# Autodesk Inventor assembly: Сборка
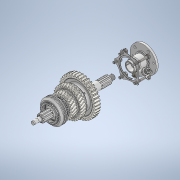
[picture p0: Inventor's stored thumbnail of the model, 180x180]
Saved by Autodesk Inventor 2021 (Build 250183000, 183)
## iProperties
Created: 2021-04-26
Part Number: Сборка
Document SubType Name: Assembly
Designer: Данил
Author: Данил
## Documents named in this file (29)
- C:\Users\Данил\Desktop\Коробка передач\Детали\Сборка.iam
- C:\Users\Данил\Desktop\Коробка передач\Детали\66-67. Картер коробки передач.ipt
- C:\Users\Данил\Desktop\Коробка передач\Детали\74. Вал первичный в сборе.iam
- C:\Users\Данил\Desktop\Коробка передач\Детали\Подшипник 180209 ГОСТ 8882-75.ipt
- C:\Users\Данил\Desktop\Коробка передач\Детали\65. Кольцо упорное подшипника.ipt
- C:\Users\Данил\Desktop\Коробка передач\Детали\76. Гайка первичного вала.ipt
- C:\Users\Данил\Desktop\Коробка передач\Детали\75. Прокладка крышки.ipt
- C:\Users\Данил\Desktop\Коробка передач\Детали\73. Крышка подшипника.ipt
- C:\Users\Данил\Desktop\Коробка передач\Детали\34. Скоба оттяжной пружины муфты.ipt
- C:\Users\Данил\Documents\Inventor\Content Center Files\R2021\ru-RU\GOST 6402-70\Шайба  8 L ГОСТ 6402-70.ipt
- C:\Users\Данил\Documents\Inventor\Content Center Files\R2021\ru-RU\Bolt GOST 7798-78\Болт M8-6g×22(S13) ГОСТ 7798-70.ipt
- C:\Users\Данил\Desktop\Коробка передач\Детали\73. Вал вторичный в сборе.iam
- C:\Users\Данил\Desktop\Коробка передач\Детали\64. Кольцо блокирующее.ipt
- C:\Users\Данил\Desktop\Коробка передач\Детали\Подшипник 307 ГОСТ 8338-75.ipt
- C:\Users\Данил\Desktop\Коробка передач\Детали\79. Кольцо стопорное.ipt
- C:\Users\Данил\Desktop\Коробка передач\Детали\74. Прокладка задней крышки.ipt
- C:\Users\Данил\Desktop\Коробка передач\Детали\76. Шестерня спидометра ведущая.ipt
- C:\Users\Данил\Desktop\Коробка передач\Детали\65. Муфта вторичного вала.ipt
- C:\Users\Данил\Desktop\Коробка передач\Детали\136. Шайба.ipt
- C:\Users\Данил\Desktop\Коробка передач\Детали\70. Крышка задняя.ipt
- C:\Users\Данил\Desktop\Коробка передач\Детали\69. Гайка крепления фланца.ipt
- C:\Users\Данил\Desktop\Коробка передач\Детали\411. Штуцер гибкого вала.ipt
- C:\Users\Данил\Desktop\Коробка передач\Детали\75. Шестерня спидометра ведомая.iam
- C:\Users\Данил\Desktop\Коробка передач\Детали\76. Стопор штуцера.ipt
- C:\Users\Данил\Documents\Inventor\Content Center Files\R2021\ru-RU\GOST 6402-70\Шайба  6 L ГОСТ 6402-70.ipt
- C:\Users\Данил\Documents\Inventor\Content Center Files\R2021\ru-RU\Bolt GOST 7798-78\Болт M6-6g×12(S10) ГОСТ 7798-70.ipt
- C:\Users\Данил\Documents\Inventor\Content Center Files\R2021\ru-RU\GOST 6402-70\Шайба  10 N ГОСТ 6402-70.ipt
- C:\Users\Данил\Documents\Inventor\Content Center Files\R2021\ru-RU\Bolt GOST 7798-78\Болт M10-6g×60(S16) ГОСТ 7798-70.ipt
- C:\Users\Данил\Documents\Inventor\Content Center Files\R2021\ru-RU\Bolt GOST 7798-78\Болт M10-6g×25(S16) ГОСТ 7798-70.ipt
## Components (41 placed, 28 different names)
1. 66-67. Картер коробки передач:1 — Совмещение:5, Совмещение:8, Совмещение:9, Совмещение:10, Совмещение:11, Совмещение:14, Совмещение:15, Совмещение:41, Совмещение:42, Совмещение:43, Совмещение:52, Совмещение:53
2. 74. Вал первичный в сборе:1 [sub-assembly] — Совмещение:1, Совмещение:2, Совмещение:5, Совмещение:6, Совмещение:13, Совмещение:36
3. Подшипник 180000 ГОСТ 8882-75 180209:1 — Совмещение:1, Совмещение:2, Совмещение:3, Совмещение:4, Совмещение:7
4. 65. Кольцо упорное подшипника:1 — Совмещение:3, Совмещение:4, Совмещение:12
5. 76. Гайка первичного вала:1 — Совмещение:6, Совмещение:7
6. 75. Прокладка крышки:1 — Совмещение:8, Совмещение:9, Совмещение:10, Совмещение:11, Совмещение:12, Совмещение:16
7. 73. Крышка подшипника:1 — Совмещение:13, Совмещение:14, Совмещение:15, Совмещение:16, Совмещение:17, Угол:1, Совмещение:18, Совмещение:23, Совмещение:24, Совмещение:25, Совмещение:26, Совмещение:27, Совмещение:28, Совмещение:35
8. 34. Скоба оттяжной пружины муфты:1 — Совмещение:17, Угол:1, Совмещение:18, Совмещение:29, Совмещение:30
9. Шайба ГОСТ 6402-70 8 L:1 — Совмещение:19, Совмещение:27, Совмещение:33
10. Болт ГОСТ 7798-70 M8-6g×22(S13):1 — Совмещение:19, Совмещение:24, Совмещение:33
11. Шайба ГОСТ 6402-70 8 L:2 — Совмещение:30, Совмещение:31
12. Болт ГОСТ 7798-70 M8-6g×22(S13):2 — Совмещение:25, Совмещение:31
13. Шайба ГОСТ 6402-70 8 L:3 — Совмещение:28, Совмещение:34
14. Болт ГОСТ 7798-70 M8-6g×22(S13):3 — Совмещение:26, Совмещение:34
15. Шайба ГОСТ 6402-70 8 L:4 — Совмещение:29, Совмещение:32
16. Болт ГОСТ 7798-70 M8-6g×22(S13):4 — Совмещение:23, Совмещение:32
17. 73. Вал вторичный в сборе:1 [sub-assembly] — Совмещение:35, Угол:2, Совмещение:37, Совмещение:38
18. 64. Кольцо блокирующее:1 — Совмещение:36, Угол:2, Совмещение:37
19. Подшипник ГОСТ 8338-75 307:1 — Совмещение:38, Совмещение:39, Совмещение:40, Совмещение:45, Совмещение:46
20. 79. Кольцо стопорное:1 — Совмещение:39, Совмещение:40, Совмещение:44
21. 74. Прокладка задней крышки:1 — Совмещение:41, Совмещение:42, Совмещение:43, Совмещение:44, Совмещение:54
22. 76. Шестерня спидометра ведущая:1 — Совмещение:45, Совмещение:46, Совмещение:47, Совмещение:48, Совмещение:49, Совмещение:51
23. 65. Муфта вторичного вала:1 — Совмещение:47, Совмещение:48, Совмещение:50
24. 136. Шайба:1 — Совмещение:49, Совмещение:50, Совмещение:55, Совмещение:56
25. 70. Крышка задняя:1 — Совмещение:51, Совмещение:52, Совмещение:53, Совмещение:54, Совмещение:58, Совмещение:61, Совмещение:64, Совмещение:67, Совмещение:70, Совмещение:72, Совмещение:74, Совмещение:76, Совмещение:80, Совмещение:81, Совмещение:82, Совмещение:86, Совмещение:87, Совмещение:88
26. 69. Гайка крепления фланца:1 — Совмещение:55, Совмещение:56
27. 411. Штуцер гибкого вала:1 — Совмещение:58, Совмещение:59, Совмещение:61, Совмещение:68, Заподлицо:1
28. 75. Шестерня спидометра ведомая:1 [sub-assembly] — Совмещение:59, Заподлицо:1
29. 76. Стопор штуцера:1 — Совмещение:66, Совмещение:67, Совмещение:68
30. Шайба ГОСТ 6402-70 6 L:1 — Совмещение:65
31. Болт ГОСТ 7798-70 M6-6g×12(S10):1 — Совмещение:64, Совмещение:65, Совмещение:66
32. Шайба ГОСТ 6402-70 10 N:1 — Совмещение:71, Совмещение:72
33. Болт ГОСТ 7798-70 M10-6g×60(S16):1 — Совмещение:70, Совмещение:71
34. Болт ГОСТ 7798-70 M10-6g×60(S16):2 — Совмещение:74, Совмещение:75
35. Шайба ГОСТ 6402-70 10 N:2 — Совмещение:75, Совмещение:76
36. Шайба ГОСТ 6402-70 10 N:3 — Совмещение:85, Совмещение:88
37. Болт ГОСТ 7798-70 M10-6g×25(S16):1 — Совмещение:80, Совмещение:85
38. Шайба ГОСТ 6402-70 10 N:4 — Совмещение:84, Совмещение:87
39. Болт ГОСТ 7798-70 M10-6g×25(S16):2 — Совмещение:81, Совмещение:84
40. Шайба ГОСТ 6402-70 10 N:5 — Совмещение:83, Совмещение:86
41. Болт ГОСТ 7798-70 M10-6g×25(S16):3 — Совмещение:82, Совмещение:83
## Relationships (90: Mate 87, Angle 2, Flush 1)
- Совмещение:1 [Mate]: 74. Вал первичный в сборе:1 ↔ Подшипник 180000 ГОСТ 8882-75 180209:1
- Совмещение:2 [Mate]: 74. Вал первичный в сборе:1 ↔ Подшипник 180000 ГОСТ 8882-75 180209:1
- Совмещение:3 [Mate]: Подшипник 180000 ГОСТ 8882-75 180209:1 ↔ 65. Кольцо упорное подшипника:1
- Совмещение:4 [Mate]: Подшипник 180000 ГОСТ 8882-75 180209:1 ↔ 65. Кольцо упорное подшипника:1
- Совмещение:5 [Mate]: 66-67. Картер коробки передач:1 ↔ 74. Вал первичный в сборе:1
- Совмещение:6 [Mate]: 74. Вал первичный в сборе:1 ↔ 76. Гайка первичного вала:1
- Совмещение:7 [Mate]: Подшипник 180000 ГОСТ 8882-75 180209:1 ↔ 76. Гайка первичного вала:1
- Совмещение:8 [Mate]: 66-67. Картер коробки передач:1 ↔ 75. Прокладка крышки:1
- Совмещение:9 [Mate]: 66-67. Картер коробки передач:1 ↔ 75. Прокладка крышки:1
- Совмещение:10 [Mate]: 66-67. Картер коробки передач:1 ↔ 75. Прокладка крышки:1
- Совмещение:11 [Mate]: 66-67. Картер коробки передач:1 ↔ 75. Прокладка крышки:1
- Совмещение:12 [Mate]: 65. Кольцо упорное подшипника:1 ↔ 75. Прокладка крышки:1
- Совмещение:13 [Mate]: 74. Вал первичный в сборе:1 ↔ 73. Крышка подшипника:1
- Совмещение:14 [Mate]: 66-67. Картер коробки передач:1 ↔ 73. Крышка подшипника:1
- Совмещение:15 [Mate]: 66-67. Картер коробки передач:1 ↔ 73. Крышка подшипника:1
- Совмещение:16 [Mate]: 75. Прокладка крышки:1 ↔ 73. Крышка подшипника:1
- Совмещение:17 [Mate]: 73. Крышка подшипника:1 ↔ 34. Скоба оттяжной пружины муфты:1
- Угол:1 [Angle] (0 deg): 73. Крышка подшипника:1 ↔ 34. Скоба оттяжной пружины муфты:1
- Совмещение:18 [Mate]: 73. Крышка подшипника:1 ↔ 34. Скоба оттяжной пружины муфты:1
- Совмещение:19 [Mate]: Шайба ГОСТ 6402-70 8 L:1 ↔ Болт ГОСТ 7798-70 M8-6g×22(S13):1
- [Mate]: Шайба ГОСТ 6402-70 8 L:2 ↔ Болт ГОСТ 7798-70 M8-6g×22(S13):2
- [Mate]: Шайба ГОСТ 6402-70 8 L:3 ↔ Болт ГОСТ 7798-70 M8-6g×22(S13):3
- [Mate]: Шайба ГОСТ 6402-70 8 L:4 ↔ Болт ГОСТ 7798-70 M8-6g×22(S13):4
- Совмещение:23 [Mate]: 73. Крышка подшипника:1 ↔ Болт ГОСТ 7798-70 M8-6g×22(S13):4
- Совмещение:24 [Mate]: 73. Крышка подшипника:1 ↔ Болт ГОСТ 7798-70 M8-6g×22(S13):1
- Совмещение:25 [Mate]: 73. Крышка подшипника:1 ↔ Болт ГОСТ 7798-70 M8-6g×22(S13):2
- Совмещение:26 [Mate]: 73. Крышка подшипника:1 ↔ Болт ГОСТ 7798-70 M8-6g×22(S13):3
- Совмещение:27 [Mate]: 73. Крышка подшипника:1 ↔ Шайба ГОСТ 6402-70 8 L:1
- Совмещение:28 [Mate]: 73. Крышка подшипника:1 ↔ Шайба ГОСТ 6402-70 8 L:3
- Совмещение:29 [Mate]: 34. Скоба оттяжной пружины муфты:1 ↔ Шайба ГОСТ 6402-70 8 L:4
- Совмещение:30 [Mate]: 34. Скоба оттяжной пружины муфты:1 ↔ Шайба ГОСТ 6402-70 8 L:2
- Совмещение:31 [Mate]: Шайба ГОСТ 6402-70 8 L:2 ↔ Болт ГОСТ 7798-70 M8-6g×22(S13):2
- Совмещение:32 [Mate]: Шайба ГОСТ 6402-70 8 L:4 ↔ Болт ГОСТ 7798-70 M8-6g×22(S13):4
- Совмещение:33 [Mate]: Шайба ГОСТ 6402-70 8 L:1 ↔ Болт ГОСТ 7798-70 M8-6g×22(S13):1
- Совмещение:34 [Mate]: Шайба ГОСТ 6402-70 8 L:3 ↔ Болт ГОСТ 7798-70 M8-6g×22(S13):3
- Совмещение:35 [Mate]: 73. Крышка подшипника:1 ↔ 73. Вал вторичный в сборе:1
- Совмещение:36 [Mate]: 74. Вал первичный в сборе:1 ↔ 64. Кольцо блокирующее:1
- Угол:2 [Angle] (0 deg): 73. Вал вторичный в сборе:1 ↔ 64. Кольцо блокирующее:1
- Совмещение:37 [Mate]: 73. Вал вторичный в сборе:1 ↔ 64. Кольцо блокирующее:1
- Совмещение:38 [Mate]: 73. Вал вторичный в сборе:1 ↔ Подшипник ГОСТ 8338-75 307:1
- Совмещение:39 [Mate]: Подшипник ГОСТ 8338-75 307:1 ↔ 79. Кольцо стопорное:1
- Совмещение:40 [Mate]: Подшипник ГОСТ 8338-75 307:1 ↔ 79. Кольцо стопорное:1
- Совмещение:41 [Mate]: 66-67. Картер коробки передач:1 ↔ 74. Прокладка задней крышки:1
- Совмещение:42 [Mate]: 66-67. Картер коробки передач:1 ↔ 74. Прокладка задней крышки:1
- Совмещение:43 [Mate]: 66-67. Картер коробки передач:1 ↔ 74. Прокладка задней крышки:1
- Совмещение:44 [Mate]: 79. Кольцо стопорное:1 ↔ 74. Прокладка задней крышки:1
- Совмещение:45 [Mate]: Подшипник ГОСТ 8338-75 307:1 ↔ 76. Шестерня спидометра ведущая:1
- Совмещение:46 [Mate]: Подшипник ГОСТ 8338-75 307:1 ↔ 76. Шестерня спидометра ведущая:1
- Совмещение:47 [Mate]: 76. Шестерня спидометра ведущая:1 ↔ 65. Муфта вторичного вала:1
- Совмещение:48 [Mate]: 76. Шестерня спидометра ведущая:1 ↔ 65. Муфта вторичного вала:1
- Совмещение:49 [Mate]: 76. Шестерня спидометра ведущая:1 ↔ 136. Шайба:1
- Совмещение:50 [Mate]: 65. Муфта вторичного вала:1 ↔ 136. Шайба:1
- Совмещение:51 [Mate]: 76. Шестерня спидометра ведущая:1 ↔ 70. Крышка задняя:1
- Совмещение:52 [Mate]: 66-67. Картер коробки передач:1 ↔ 70. Крышка задняя:1
- Совмещение:53 [Mate]: 66-67. Картер коробки передач:1 ↔ 70. Крышка задняя:1
- Совмещение:54 [Mate]: 74. Прокладка задней крышки:1 ↔ 70. Крышка задняя:1
- Совмещение:55 [Mate]: 136. Шайба:1 ↔ 69. Гайка крепления фланца:1
- Совмещение:56 [Mate]: 136. Шайба:1 ↔ 69. Гайка крепления фланца:1
- [Mate]: 411. Штуцер гибкого вала:1 ↔ 75. Шестерня спидометра ведомая:1
- Совмещение:58 [Mate]: 70. Крышка задняя:1 ↔ 411. Штуцер гибкого вала:1
- Совмещение:59 [Mate]: 411. Штуцер гибкого вала:1 ↔ 75. Шестерня спидометра ведомая:1
- Совмещение:61 [Mate]: 70. Крышка задняя:1 ↔ 411. Штуцер гибкого вала:1
- [Mate]: 76. Стопор штуцера:1 ↔ Шайба ГОСТ 6402-70 6 L:1
- [Mate]: Шайба ГОСТ 6402-70 6 L:1 ↔ Болт ГОСТ 7798-70 M6-6g×12(S10):1
- Совмещение:64 [Mate]: 70. Крышка задняя:1 ↔ Болт ГОСТ 7798-70 M6-6g×12(S10):1
- Совмещение:65 [Mate]: Шайба ГОСТ 6402-70 6 L:1 ↔ Болт ГОСТ 7798-70 M6-6g×12(S10):1
- Совмещение:66 [Mate]: 76. Стопор штуцера:1 ↔ Болт ГОСТ 7798-70 M6-6g×12(S10):1
- Совмещение:67 [Mate]: 70. Крышка задняя:1 ↔ 76. Стопор штуцера:1
- Совмещение:68 [Mate]: 411. Штуцер гибкого вала:1 ↔ 76. Стопор штуцера:1
- Заподлицо:1 [Flush] (-5 mm): 411. Штуцер гибкого вала:1 ↔ 75. Шестерня спидометра ведомая:1
- [Mate]: Шайба ГОСТ 6402-70 10 N:1 ↔ Болт ГОСТ 7798-70 M10-6g×60(S16):1
- Совмещение:70 [Mate]: 70. Крышка задняя:1 ↔ Болт ГОСТ 7798-70 M10-6g×60(S16):1
- Совмещение:71 [Mate]: Шайба ГОСТ 6402-70 10 N:1 ↔ Болт ГОСТ 7798-70 M10-6g×60(S16):1
- Совмещение:72 [Mate]: 70. Крышка задняя:1 ↔ Шайба ГОСТ 6402-70 10 N:1
- [Mate]: Болт ГОСТ 7798-70 M10-6g×60(S16):2 ↔ Шайба ГОСТ 6402-70 10 N:2
- Совмещение:74 [Mate]: 70. Крышка задняя:1 ↔ Болт ГОСТ 7798-70 M10-6g×60(S16):2
- Совмещение:75 [Mate]: Болт ГОСТ 7798-70 M10-6g×60(S16):2 ↔ Шайба ГОСТ 6402-70 10 N:2
- Совмещение:76 [Mate]: 70. Крышка задняя:1 ↔ Шайба ГОСТ 6402-70 10 N:2
- [Mate]: Шайба ГОСТ 6402-70 10 N:3 ↔ Болт ГОСТ 7798-70 M10-6g×25(S16):1
- [Mate]: Шайба ГОСТ 6402-70 10 N:4 ↔ Болт ГОСТ 7798-70 M10-6g×25(S16):2
- [Mate]: Шайба ГОСТ 6402-70 10 N:5 ↔ Болт ГОСТ 7798-70 M10-6g×25(S16):3
- Совмещение:80 [Mate]: 70. Крышка задняя:1 ↔ Болт ГОСТ 7798-70 M10-6g×25(S16):1
- Совмещение:81 [Mate]: 70. Крышка задняя:1 ↔ Болт ГОСТ 7798-70 M10-6g×25(S16):2
- Совмещение:82 [Mate]: 70. Крышка задняя:1 ↔ Болт ГОСТ 7798-70 M10-6g×25(S16):3
- Совмещение:83 [Mate]: Шайба ГОСТ 6402-70 10 N:5 ↔ Болт ГОСТ 7798-70 M10-6g×25(S16):3
- Совмещение:84 [Mate]: Шайба ГОСТ 6402-70 10 N:4 ↔ Болт ГОСТ 7798-70 M10-6g×25(S16):2
- Совмещение:85 [Mate]: Шайба ГОСТ 6402-70 10 N:3 ↔ Болт ГОСТ 7798-70 M10-6g×25(S16):1
- Совмещение:86 [Mate]: 70. Крышка задняя:1 ↔ Шайба ГОСТ 6402-70 10 N:5
- Совмещение:87 [Mate]: 70. Крышка задняя:1 ↔ Шайба ГОСТ 6402-70 10 N:4
- Совмещение:88 [Mate]: 70. Крышка задняя:1 ↔ Шайба ГОСТ 6402-70 10 N:3
## Named parameters: d21_d20 = 0 mm, d22_d20 = 0 mm, d23_d20 = 0 mm, d81_d181 = 0 mm, d82_d181 = 0 mm
